# Autodesk Inventor assembly: claws_endeffector
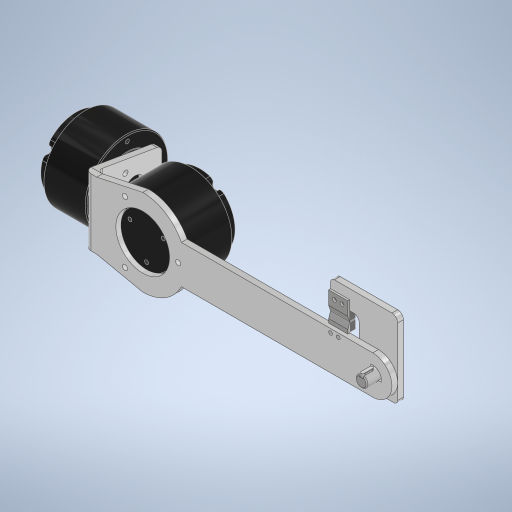
[picture p0: Inventor's stored thumbnail of the model, 512x512]
Saved by Autodesk Inventor 2024 (Build 280153000, 153)
## iProperties
Created: 2025-02-08
Part Number: claws_endeffector
Document SubType Name: Assembly
Designer: 1412z
Author: 1412z
## Documents named in this file (8)
- C:\Users\1412z\OneDrive\デスクトップ\rdclab\harvesting_robot\tsutsui's_endeffector\claws_endeffector.iam
- C:\Users\1412z\OneDrive\デスクトップ\rdclab\harvesting_robot\tsutsui's_endeffector\motor_holder\motor_holder_1.ipt
- C:\Users\1412z\OneDrive\デスクトップ\rdclab\harvesting_robot\tsutsui's_endeffector\GIM3505-08\GIM3505-8_with-driver.ipt
- C:\Users\1412z\OneDrive\デスクトップ\rdclab\harvesting_robot\tsutsui's_endeffector\misumi\SSFHKR6-15-KA0-A6-KB9-B6_Autodesk_Inventor_2024_20250208\AIS2024\SSFHKR6-15-KA0-A6-KB9-B6_s.ipt
- C:\Users\1412z\OneDrive\デスクトップ\rdclab\harvesting_robot\tsutsui's_endeffector\misumi\KESS2-6_Autodesk_Inventor_2024_20250208\KESS2-6.ipt
- C:\Users\1412z\OneDrive\デスクトップ\rdclab\harvesting_robot\tsutsui's_endeffector\cutter_part\cutter_holder.ipt
- C:\Users\1412z\OneDrive\デスクトップ\rdclab\harvesting_robot\tsutsui's_endeffector\cutter_part\cutter.ipt
- C:\Users\1412z\OneDrive\デスクトップ\rdclab\harvesting_robot\tsutsui's_endeffector\cutter_part\sponge.ipt
## Components (11 placed, 7 different names)
1. motor_holder_1:1 — 回転:1, 回転:2, 回転:3, 回転:4, 回転:7, 回転:8, 回転:11, 回転:12
2. GIM3505-8_with-driver:1 — 回転:1, 回転:2
3. GIM3505-8_with-driver:2 — 回転:3, 回転:4
4. SSFHKR6-15-KA0-A6-KB9-B6_s:1 — 回転:7, 回転:5, 回転:6
5. KESS2-6:1 — 回転:5
6. KESS2-6:2 — 回転:6
7. cutter_holder:1 — 回転:8, 回転:9, 回転:10
8. cutter:1 — 回転:9, 回転:10, リジッド:1
9. cutter:2 — 回転:11, 回転:12, リジッド:2
10. sponge:1 — リジッド:2
11. sponge:2 — リジッド:1
## Relationships (14: RevoluteJoint 12, WeldJoint 2)
- 回転:1 [RevoluteJoint]: motor_holder_1:1 ↔ GIM3505-8_with-driver:1
- 回転:2 [RevoluteJoint]: motor_holder_1:1 ↔ GIM3505-8_with-driver:1
- 回転:3 [RevoluteJoint]: motor_holder_1:1 ↔ GIM3505-8_with-driver:2
- 回転:4 [RevoluteJoint]: motor_holder_1:1 ↔ GIM3505-8_with-driver:2
- 回転:7 [RevoluteJoint] (-1.5 mm): motor_holder_1:1 ↔ SSFHKR6-15-KA0-A6-KB9-B6_s:1
- 回転:5 [RevoluteJoint]: SSFHKR6-15-KA0-A6-KB9-B6_s:1 ↔ KESS2-6:1
- 回転:6 [RevoluteJoint]: SSFHKR6-15-KA0-A6-KB9-B6_s:1 ↔ KESS2-6:2
- 回転:8 [RevoluteJoint]: motor_holder_1:1 ↔ cutter_holder:1
- 回転:9 [RevoluteJoint]: cutter_holder:1 ↔ cutter:1
- 回転:10 [RevoluteJoint]: cutter_holder:1 ↔ cutter:1
- 回転:11 [RevoluteJoint]: motor_holder_1:1 ↔ cutter:2
- 回転:12 [RevoluteJoint]: motor_holder_1:1 ↔ cutter:2
- リジッド:1 [WeldJoint] (2.5 mm): cutter:1 ↔ sponge:2
- リジッド:2 [WeldJoint] (-2.5 mm): cutter:2 ↔ sponge:1
